# Autodesk Inventor assembly: Cơ cấu gạt cốc
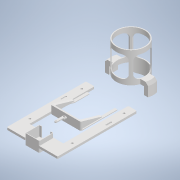
[picture p0: Inventor's stored thumbnail of the model, 180x180]
Saved by Autodesk Inventor 2020 (Build 240168000, 168)
## iProperties
Created: 2022-11-23
Part Number: Cơ cấu gạt cốc
Document SubType Name: Assembly
Designer: ADMIN
Author: ADMIN
## Documents named in this file (6)
- D:\Do-an-tot-nghiep\Inventor\Cơ cấu gạt cốc.iam
- D:\Do-an-tot-nghiep\Inventor\Hộp đựng động cơ.ipt
- D:\Do-an-tot-nghiep\Inventor\Khay đựng cốc.ipt
- D:\Do-an-tot-nghiep\Inventor\Khay gạt cốc.ipt
- D:\Do-an-tot-nghiep\Inventor\tay quay.ipt
- C:\Users\ADMIN\Documents\Inventor\Content Center Files\R2020\en-US\ISO 2338(2)\ISO 2338 - 4 h8 x 8.ipt
## Components (5 placed, 5 different names)
1. Hộp đựng động cơ:1 — Mate:1, Mate:2
2. Khay đựng cốc:1 — Mate:1
3. Khay gạt cốc:1 — Mate:2, Mate:3, Mate:4
4. tay quay:1 — Mate:3, Mate:4, Mate:5
5. ISO 2338 4 h8 x 8:1 — Mate:5
## Relationships (5: Mate 5)
- Mate:1: Hộp đựng động cơ:1 ↔ Khay đựng cốc:1
- Mate:2: Hộp đựng động cơ:1 ↔ Khay gạt cốc:1
- Mate:3: Khay gạt cốc:1 ↔ tay quay:1
- Mate:4: Khay gạt cốc:1 ↔ tay quay:1
- Mate:5: tay quay:1 ↔ ISO 2338 4 h8 x 8:1
